# Autodesk Inventor assembly: ScanningCoils
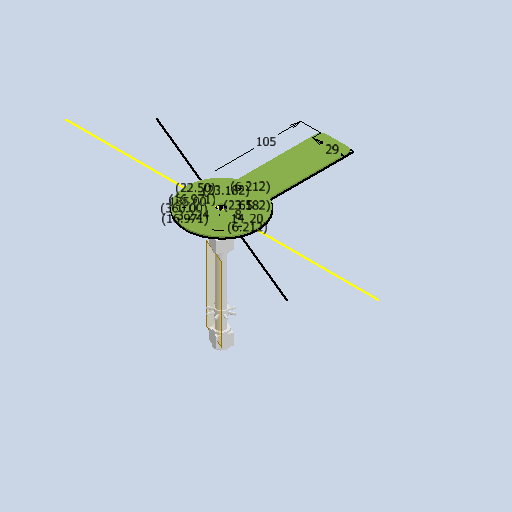
[picture p0: Inventor's stored thumbnail of the model, 512x512]
Saved by Autodesk Inventor 2023 (Build 270158000, 158)
## iProperties
Created: 2022-04-26
Part Number: ScanningCoils
Document SubType Name: Assembly
Designer: vmiguel
Author: vmiguel
## Documents named in this file (3)
- P:\SEM-Mechanical\ScanningCoils.iam
- P:\SEM-Mechanical\038.ipt
- P:\SEM-Mechanical\039.ipt
## Components (2 placed, 2 different names)
1. 038:1 — Flush:1, Flush:2, Flush:3, Flush:4, Mate:1, Angle:1
2. 039:1 — Flush:4, Mate:1, Angle:1
## Relationships (6: Flush 4, Mate 1, Angle 1)
- Flush:1: 038:1
- Flush:2: 038:1
- Flush:3: 038:1
- Flush:4: 038:1 ↔ 039:1
- Mate:1: 038:1 ↔ 039:1
- Angle:1 (0 deg): 038:1 ↔ 039:1
